# Autodesk Inventor assembly: LV Base +  Cap
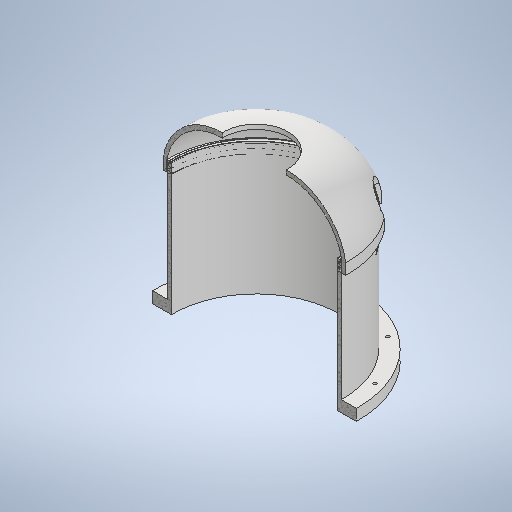
[picture p0: Inventor's stored thumbnail of the model, 512x512]
Saved by Autodesk Inventor 2025 (Build 290162000, 162)
## iProperties
Created: 2025-07-16
Part Number: LV Base +  Cap
Document SubType Name: Assembly
Designer: mumin
Author: mumin
## Documents named in this file (3)
- C:\GitHub\In-situ-monitoring-of-powder-bed-fusion-additive-manufacturing\system_development\Orichalcum\v0.3\LV Base +  Cap.iam
- C:\GitHub\In-situ-monitoring-of-powder-bed-fusion-additive-manufacturing\system_development\Orichalcum\v0.3\Cylinder Housing_cap.ipt
- C:\GitHub\In-situ-monitoring-of-powder-bed-fusion-additive-manufacturing\system_development\Orichalcum\v0.3\Cylinder Housing_base.ipt
## Components (2 placed, 2 different names)
1. Cylinder Housing_base:1 — Insert:1
2. Cylinder Housing_cap:1 — Insert:1
## Relationships (1: Insert 1)
- Insert:1: Cylinder Housing_base:1 ↔ Cylinder Housing_cap:1
